# Autodesk Inventor assembly: Fan 6020
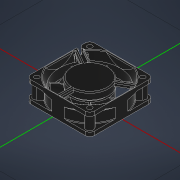
[picture p0: Inventor's stored thumbnail of the model, 180x180]
Saved by Autodesk Inventor 2022.2 (Build 262287010, 287A)
## iProperties
Created: 2022-03-13
Part Number: Fan 6020
Document SubType Name: Assembly
Designer: sleib
Author: sleib
## Documents named in this file (3)
- C:\Users\sleib\Projekte\Voron-2\CAD\Inventor\Fan 6020.iam
- C:\Users\sleib\Projekte\Voron-2\CAD\Inventor\Fan Housing 6020.ipt
- C:\Users\sleib\Projekte\Voron-2\CAD\Inventor\Fan Impeller 6020.ipt
## Components (2 placed, 2 different names)
1. Fan Housing 6020:1 — Passend:1, Passend:2
2. Fan Impeller 6020:1 — Passend:1, Passend:2
## Relationships (2: Mate 2)
- Passend:1 [Mate]: Fan Housing 6020:1 ↔ Fan Impeller 6020:1
- Passend:2 [Mate] (2 mm): Fan Housing 6020:1 ↔ Fan Impeller 6020:1
